# Autodesk Inventor assembly: System_Box_Assembly1
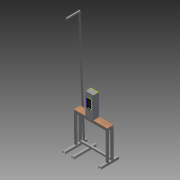
[picture p0: Inventor's stored thumbnail of the model, 180x180]
Saved by Autodesk Inventor 2015 SP2 (Build 190223200, 223)
## iProperties
Created: 2017-05-28
Part Number: System_Box_Assembly1
Document SubType Name: Assembly
Designer: MehariK
_SolveAssemblyDoc: Frame Generator Solve Assembly
_Version: 15.0.0
Author: MehariK
## Documents named in this file (14)
- H:\KIC\Theme Study B\Prototype\3D design\System_Box_Assembly1.iam
- H:\KIC\Theme Study B\Prototype\3D design\System_Box_Part1.ipt
- H:\KIC\Theme Study B\Prototype\3D design\System_Box_Assembly1\Frame\Frame0001.iam
- H:\KIC\Theme Study B\Prototype\3D design\System_Box_Top_and_Bottom_Cover.ipt
- H:\KIC\Theme Study B\Prototype\3D design\System_Box_Three Side Cover.ipt
- H:\KIC\Theme Study B\Prototype\3D design\Bench_Assemble1.iam
- H:\KIC\Theme Study B\Prototype\3D design\Horizontal Kiosk Stand ISO 4019 - 50x50x2 - 400.ipt
- H:\KIC\Theme Study B\Prototype\3D design\Horizontal Kiosk Stand ISO 4019 - 50x50x2 - 500.ipt
- H:\KIC\Theme Study B\Prototype\3D design\Height Bar ISO 4019 - 30x30x3 - 2500.ipt
- H:\KIC\Theme Study B\Prototype\3D design\Height Top Horizontal Bar ISO 4019 - 30x30x3 - 2500.ipt
- H:\KIC\Theme Study B\Prototype\3D design\Top Cover for the EHealth Kiosk.ipt
- H:\KIC\Theme Study B\Prototype\3D design\Top Cover for the EHealth Kiosk Left Side.ipt
- H:\KIC\Theme Study B\Prototype\3D design\Raspberry PI standard display Part.ipt
- H:\KIC\Theme Study B\Prototype\3D design\Logo Kiosk.ipt
## Components (15 placed, 13 different names)
1. System_Box_Part1:1
2. Frame0001:1 [sub-assembly] — Mate:1, Mate:2, Mate:3, Mate:4, Mate:5, Mate:6
3. System_Box_Top_and_Bottom_Cover:1 — Mate:1, Mate:2
4. System_Box_Top_and_Bottom_Cover:2 — Mate:3, Mate:4, Mate:8
5. System_Box_Three Side Cover:1 — Mate:5, Mate:6, Mate:7, Mate:20
6. Bench_Assemble1:1 [sub-assembly] — Mate:7, Mate:8, Mate:10, Mate:11, Mate:12, Mate:15, Mate:17, Mate:18, Mate:19
7. Horizontal Kiosk Stand ISO 4019 - 50x50x2 - 400:2 — Mate:10
8. Horizontal Kiosk Stand ISO 4019 - 50x50x2 - 500:1 — Mate:11, Mate:16
9. Horizontal Kiosk Stand ISO 4019 - 50x50x2 - 500:2 — Mate:12
10. Height Bar ISO 4019 - 30x30x3 - 2500:1 — Mate:13, Mate:14, Mate:15, Mate:16
11. Height Top Horizontal Bar ISO 4019 - 30x30x3 - 2500:1 — Mate:13, Mate:14
12. Top Cover for the EHealth Kiosk:1 — Mate:17
13. Top Cover for the EHealth Kiosk Left Side:1 — Mate:18, Mate:19
14. Raspberry PI standard display Part:1 — Mate:20, Mate:21
15. Logo Kiosk:1 — Mate:21
## Relationships (20: Mate 20)
- Mate:1: Frame0001:1 ↔ System_Box_Top_and_Bottom_Cover:1
- Mate:2: Frame0001:1 ↔ System_Box_Top_and_Bottom_Cover:1
- Mate:3: Frame0001:1 ↔ System_Box_Top_and_Bottom_Cover:2
- Mate:4: Frame0001:1 ↔ System_Box_Top_and_Bottom_Cover:2
- Mate:5: Frame0001:1 ↔ System_Box_Three Side Cover:1
- Mate:6: Frame0001:1 ↔ System_Box_Three Side Cover:1
- Mate:7: System_Box_Three Side Cover:1 ↔ Bench_Assemble1:1
- Mate:8: System_Box_Top_and_Bottom_Cover:2 ↔ Bench_Assemble1:1
- Mate:10: Bench_Assemble1:1 ↔ Horizontal Kiosk Stand ISO 4019 - 50x50x2 - 400:2
- Mate:11: Bench_Assemble1:1 ↔ Horizontal Kiosk Stand ISO 4019 - 50x50x2 - 500:1
- Mate:12: Bench_Assemble1:1 ↔ Horizontal Kiosk Stand ISO 4019 - 50x50x2 - 500:2
- Mate:13: Height Bar ISO 4019 - 30x30x3 - 2500:1 ↔ Height Top Horizontal Bar ISO 4019 - 30x30x3 - 2500:1
- Mate:14: Height Bar ISO 4019 - 30x30x3 - 2500:1 ↔ Height Top Horizontal Bar ISO 4019 - 30x30x3 - 2500:1
- Mate:15: Bench_Assemble1:1 ↔ Height Bar ISO 4019 - 30x30x3 - 2500:1
- Mate:16: Horizontal Kiosk Stand ISO 4019 - 50x50x2 - 500:1 ↔ Height Bar ISO 4019 - 30x30x3 - 2500:1
- Mate:17: Bench_Assemble1:1 ↔ Top Cover for the EHealth Kiosk:1
- Mate:18: Bench_Assemble1:1 ↔ Top Cover for the EHealth Kiosk Left Side:1
- Mate:19: Bench_Assemble1:1 ↔ Top Cover for the EHealth Kiosk Left Side:1
- Mate:20: System_Box_Three Side Cover:1 ↔ Raspberry PI standard display Part:1
- Mate:21: Raspberry PI standard display Part:1 ↔ Logo Kiosk:1
